# Autodesk Inventor assembly: PneumaticWheel_am-0970-2
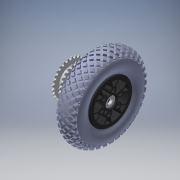
[picture p0: Inventor's stored thumbnail of the model, 180x180]
Saved by Autodesk Inventor 2016 (Build 200138000, 138)
## iProperties
Created: 2011-11-15
Part Number: PneumaticWheel_am-0970-2
Description: STEP AP214
Document SubType Name: Assembly
Designer: gus
Mass: 728.217 g
Surface Area: 2848.92 cm^2
Volume: 557.085 cm^3
Density: 1.30719 g/cm^3
Sending System: SolidWorks 2010
Preprocessor: SwSTEP 2.0
Title: Pneumatic Wheel.STEP
Author: Mark
Revision Number: ANY
## Documents named in this file (7)
- \\Mac\Home\Desktop\2016 robot cad\chassis\PneumaticWheel_am-0970-2.iam
- \\Mac\Home\Desktop\2016 robot cad\chassis\Tire.ipt
- \\Mac\Home\Desktop\2016 robot cad\chassis\Pneumatic Hub.iam
- \\Mac\Home\Desktop\2016 robot cad\chassis\spacer.ipt
- \\Mac\Home\Desktop\2016 robot cad\chassis\shaftcollar.ipt
- \\Mac\Home\Desktop\2016 robot cad\chassis\28tsprocket.ipt
- \\Mac\Home\Desktop\2016 robot cad\roller wheels\bearing.ipt
## Components (9 placed, 6 different names)
1. Tire_1 — Cylindrical:2, Rigid:1
2. Pneumatic Hub_3 [sub-assembly] — Cylindrical:2, Rigid:1, Rotational:1, Rotational:3, Mate:13, Mate:14, Mate:15
3. shaftcollar:1 — Rotational:1
4. shaftcollar:2 — Rotational:2
5. 28tsprocket:1 — Mate:7, Mate:8, Mate:9, Mate:16
6. 28tsprocket:2 — Mate:10, Mate:11, Mate:12, Mate:17, Mate:18
7. spacer:1 — Mate:7, Mate:8, Mate:9, Mate:10, Mate:11, Mate:12, Rotational:2
8. spacer:2 — Mate:13, Mate:14, Mate:15, Mate:16, Mate:17, Mate:18
9. bearing:1 — Rotational:3
## Relationships (17: Mate 12, RevoluteJoint 3, CylindricalJoint 1, WeldJoint 1)
- Cylindrical:2: Tire_1 ↔ Pneumatic Hub_3
- Rigid:1 [WeldJoint]: Tire_1 ↔ Pneumatic Hub_3
- Rotational:1 [RevoluteJoint]: Pneumatic Hub_3 ↔ shaftcollar:1
- Mate:7: 28tsprocket:1 ↔ spacer:1
- Mate:8: 28tsprocket:1 ↔ spacer:1
- Mate:9: 28tsprocket:1 ↔ spacer:1
- Mate:10: 28tsprocket:2 ↔ spacer:1
- Mate:11: 28tsprocket:2 ↔ spacer:1
- Mate:12: 28tsprocket:2 ↔ spacer:1
- Rotational:2 [RevoluteJoint]: shaftcollar:2 ↔ spacer:1
- Rotational:3 [RevoluteJoint]: Pneumatic Hub_3 ↔ bearing:1
- Mate:13: Pneumatic Hub_3 ↔ spacer:2
- Mate:14: Pneumatic Hub_3 ↔ spacer:2
- Mate:15: Pneumatic Hub_3 ↔ spacer:2
- Mate:16: 28tsprocket:1 ↔ spacer:2
- Mate:17: 28tsprocket:2 ↔ spacer:2
- Mate:18: 28tsprocket:2 ↔ spacer:2
